# Autodesk Inventor assembly: LINEAR ACTUATOR
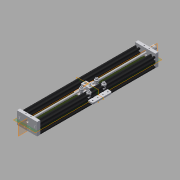
[picture p0: Inventor's stored thumbnail of the model, 180x180]
Saved by Autodesk Inventor 2016 (Build 200138000, 138)
## iProperties
Created: 2023-12-03
Part Number: LINEAR ACTUATOR
Document SubType Name: Assembly
Designer: Riskinova Oktavia
Author: Riskinova Oktavia
## Documents named in this file (33)
- D:\PROJECT NOVA 2021-2022\PBLMK-041\NEW KONSEP\LINEAR ACTUATOR.iam
- D:\PROJECT NOVA 2021-2022\PBLMK-041\PBLMK-041\Solid33.ipt
- D:\PROJECT NOVA 2021-2022\PBLMK-041\PBLMK-041\Solid45.ipt
- D:\PROJECT NOVA 2021-2022\PBLMK-041\PBLMK-041\Solid39.ipt
- D:\PROJECT NOVA 2021-2022\PBLMK-041\PBLMK-041\Solid41.ipt
- D:\PROJECT NOVA 2021-2022\PBLMK-041\PBLMK-041\Solid43.ipt
- D:\PROJECT NOVA 2021-2022\PBLMK-041\PBLMK-041\Solid44.ipt
- D:\PROJECT NOVA 2021-2022\PBLMK-041\PBLMK-041\Solid57.ipt
- D:\PROJECT NOVA 2021-2022\PBLMK-041\PBLMK-041\Solid58.ipt
- D:\PROJECT NOVA 2021-2022\PBLMK-041\PBLMK-041\Solid31.ipt
- D:\PROJECT NOVA 2021-2022\PBLMK-041\PBLMK-041\Solid32.ipt
- D:\PROJECT NOVA 2021-2022\PBLMK-041\PBLMK-041\Solid1.ipt
- D:\PROJECT NOVA 2021-2022\PBLMK-041\PBLMK-041\Solid53.ipt
- D:\PROJECT NOVA 2021-2022\PBLMK-041\PBLMK-041\Solid54.ipt
- D:\PROJECT NOVA 2021-2022\PBLMK-041\PBLMK-041\Solid55.ipt
- D:\PROJECT NOVA 2021-2022\PBLMK-041\PBLMK-041\Solid56.ipt
- D:\PROJECT NOVA 2021-2022\PBLMK-041\PBLMK-041\Solid49.ipt
- D:\PROJECT NOVA 2021-2022\PBLMK-041\PBLMK-041\Solid16.ipt
- D:\PROJECT NOVA 2021-2022\PBLMK-041\PBLMK-041\Solid15.ipt
- D:\PROJECT NOVA 2021-2022\PBLMK-041\PBLMK-041\Solid14.ipt
- D:\PROJECT NOVA 2021-2022\PBLMK-041\PBLMK-041\Solid13.ipt
- D:\PROJECT NOVA 2021-2022\PBLMK-041\PBLMK-041\Solid12.ipt
- D:\PROJECT NOVA 2021-2022\PBLMK-041\PBLMK-041\Solid11.ipt
- D:\PROJECT NOVA 2021-2022\PBLMK-041\PBLMK-041\Solid10.ipt
- D:\PROJECT NOVA 2021-2022\PBLMK-041\PBLMK-041\Solid64.ipt
- D:\PROJECT NOVA 2021-2022\PBLMK-041\PBLMK-041\Solid63.ipt
- D:\PROJECT NOVA 2021-2022\PBLMK-041\PBLMK-041\Solid62.ipt
- D:\PROJECT NOVA 2021-2022\PBLMK-041\PBLMK-041\Solid61.ipt
- D:\PROJECT NOVA 2021-2022\PBLMK-041\PBLMK-041\Solid46.ipt
- D:\PROJECT NOVA 2021-2022\PBLMK-041\PBLMK-041\Solid42.ipt
- D:\PROJECT NOVA 2021-2022\PBLMK-041\PBLMK-041\Solid40.ipt
- D:\PROJECT NOVA 2021-2022\PBLMK-041\PBLMK-041\Solid38.ipt
- D:\PROJECT NOVA 2021-2022\PBLMK-041\PBLMK-041\Solid34.ipt
## Components (59 placed, 32 different names)
1. Solid33:1
2. Solid45:1 — Flush:5
3. Solid39:1
4. Solid41:1
5. Solid43:1
6. Solid44:1 — Mate:94, Mate:95, Mate:96, Mate:97
7. Solid57:1
8. Solid58:1
9. Solid31:1
10. Solid32:1 — Flush:5
11. Solid1:1
12. Solid53:1
13. Solid54:1
14. Solid55:1
15. Solid56:1
16. Solid49:1
17. Solid16:1
18. Solid15:1
19. Solid14:1
20. Solid13:1
21. Solid12:1
22. Solid11:1
23. Solid10:1
24. Solid64:1
25. Solid63:1
26. Solid62:1
27. Solid61:1
28. Solid46:1
29. Solid42:1
30. Solid40:1
31. Solid38:1
32. Solid34:1
33. Solid49:2
34. Solid16:2
35. Solid15:2
36. Solid14:2
37. Solid13:2
38. Solid12:2
39. Solid11:2
40. Solid10:2
41. Solid49:3
42. Solid16:3
43. Solid15:3
44. Solid14:3
45. Solid13:3
46. Solid12:3
47. Solid11:3
48. Solid10:3
49. Solid49:4
50. Solid16:4
51. Solid15:4
52. Solid14:4
53. Solid13:4
54. Solid12:4
55. Solid11:4
56. Solid10:4
57. Solid1:2
58. Solid58:2 — Mate:94, Mate:96
59. Solid58:3 — Mate:95, Mate:97
## Relationships (111: Mate 91, RevoluteJoint 16, Flush 4)
- [Mate]: Solid33:1 ↔ Solid31:1
- [Mate]: Solid45:1 ↔ Solid31:1
- [Mate]: Solid31:1 ↔ Solid54:1
- [Mate]: Solid31:1 ↔ Solid53:1
- [Mate]: Solid54:1 ↔ Solid55:1
- [Mate]: Solid53:1 ↔ Solid56:1
- [Mate]: Solid31:1 ↔ Solid56:1
- [Mate]: Solid31:1 ↔ Solid55:1
- [Mate]: Solid32:1 ↔ Solid53:1
- [Mate]: Solid32:1 ↔ Solid54:1
- [RevoluteJoint]: Solid16:1 ↔ Solid14:1
- [Mate]: Solid14:1 ↔ Solid12:1
- [Mate]: Solid14:1 ↔ Solid13:1
- [Mate]: Solid16:1 ↔ Solid11:1
- [RevoluteJoint]: Solid14:1 ↔ Solid13:1
- [Mate]: Solid15:1 ↔ Solid13:1
- [RevoluteJoint]: Solid15:1 ↔ Solid13:1
- [RevoluteJoint]: Solid15:1 ↔ Solid12:1
- [Mate]: Solid12:1 ↔ Solid10:1
- [Mate]: Solid49:1 ↔ Solid15:1
- [Mate]: Solid16:1 ↔ Solid11:1
- [Mate] (2 mm): Solid49:1 ↔ Solid10:1
- [Mate]: Solid12:1 ↔ Solid10:1
- [RevoluteJoint]: Solid16:2 ↔ Solid14:2
- [Mate]: Solid14:2 ↔ Solid12:2
- [Mate]: Solid14:2 ↔ Solid13:2
- [Mate]: Solid16:2 ↔ Solid11:2
- [RevoluteJoint]: Solid14:2 ↔ Solid13:2
- [Mate]: Solid15:2 ↔ Solid13:2
- [RevoluteJoint]: Solid15:2 ↔ Solid13:2
- [RevoluteJoint]: Solid15:2 ↔ Solid12:2
- [Mate]: Solid12:2 ↔ Solid10:2
- [Mate]: Solid49:2 ↔ Solid15:2
- [Mate]: Solid16:2 ↔ Solid11:2
- [Mate] (2 mm): Solid49:2 ↔ Solid10:2
- [Mate]: Solid12:2 ↔ Solid10:2
- [RevoluteJoint]: Solid16:3 ↔ Solid14:3
- [Mate]: Solid14:3 ↔ Solid12:3
- [Mate]: Solid14:3 ↔ Solid13:3
- [Mate]: Solid16:3 ↔ Solid11:3
- [RevoluteJoint]: Solid14:3 ↔ Solid13:3
- [Mate]: Solid15:3 ↔ Solid13:3
- [RevoluteJoint]: Solid15:3 ↔ Solid13:3
- [RevoluteJoint]: Solid15:3 ↔ Solid12:3
- [Mate]: Solid12:3 ↔ Solid10:3
- [Mate]: Solid49:3 ↔ Solid15:3
- [Mate]: Solid16:3 ↔ Solid11:3
- [Mate] (2 mm): Solid49:3 ↔ Solid10:3
- [Mate]: Solid12:3 ↔ Solid10:3
- [RevoluteJoint]: Solid16:4 ↔ Solid14:4
- [Mate]: Solid14:4 ↔ Solid12:4
- [Mate]: Solid14:4 ↔ Solid13:4
- [Mate]: Solid16:4 ↔ Solid11:4
- [RevoluteJoint]: Solid14:4 ↔ Solid13:4
- [Mate]: Solid15:4 ↔ Solid13:4
- [RevoluteJoint]: Solid15:4 ↔ Solid13:4
- [RevoluteJoint]: Solid15:4 ↔ Solid12:4
- [Mate]: Solid12:4 ↔ Solid10:4
- [Mate]: Solid49:4 ↔ Solid15:4
- [Mate]: Solid16:4 ↔ Solid11:4
- [Mate] (2 mm): Solid49:4 ↔ Solid10:4
- [Mate]: Solid12:4 ↔ Solid10:4
- [Mate]: Solid32:1 ↔ Solid10:1
- [Mate]: Solid32:1 ↔ Solid49:1
- [Mate]: Solid32:1 ↔ Solid49:2
- [Mate]: Solid32:1 ↔ Solid49:2
- [Mate]: Solid32:1 ↔ Solid49:3
- [Mate]: Solid32:1 ↔ Solid49:4
- [Mate]: Solid32:1 ↔ Solid49:3
- [Mate]: Solid32:1 ↔ Solid49:4
- [Mate]: Solid54:1 ↔ Solid1:2
- [Mate]: Solid1:1 ↔ Solid53:1
- [Mate]: Solid32:1 ↔ Solid1:1
- [Mate]: Solid32:1 ↔ Solid1:2
- [Mate]: Solid31:1 ↔ Solid1:1
- [Mate]: Solid33:1 ↔ Solid46:1
- [Mate]: Solid33:1 ↔ Solid34:1
- [Mate]: Solid46:1 ↔ Solid34:1
- [Flush]: Solid33:1 ↔ Solid34:1
- [Mate]: Solid46:1 ↔ Solid42:1
- [Mate]: Solid33:1 ↔ Solid40:1
- [Mate]: Solid42:1 ↔ Solid40:1
- [Mate]: Solid33:1 ↔ Solid38:1
- [Mate]: Solid40:1 ↔ Solid38:1
- [Mate]: Solid45:1 ↔ Solid46:1
- [Flush]: Solid45:1 ↔ Solid46:1
- [Mate]: Solid33:1 ↔ Solid39:1
- [Mate]: Solid33:1 ↔ Solid43:1
- [Mate]: Solid33:1 ↔ Solid41:1
- [Mate]: Solid39:1 ↔ Solid41:1
- [Mate]: Solid41:1 ↔ Solid43:1
- [Mate]: Solid45:1 ↔ Solid44:1
- [Flush]: Solid45:1 ↔ Solid44:1
- [Mate]: Solid43:1 ↔ Solid44:1
- [Mate]: Solid44:1 ↔ Solid57:1
- [Mate]: Solid44:1 ↔ Solid58:1
- [Mate]: Solid44:1 ↔ Solid57:1
- [Mate]: Solid44:1 ↔ Solid58:1
- [Mate]: Solid61:1 ↔ Solid46:1
- [Mate]: Solid62:1 ↔ Solid46:1
- [Mate]: Solid63:1 ↔ Solid46:1
- [Mate]: Solid64:1 ↔ Solid46:1
- [Mate]: Solid61:1 ↔ Solid46:1
- [Mate]: Solid63:1 ↔ Solid46:1
- [Mate]: Solid64:1 ↔ Solid46:1
- [Mate]: Solid62:1 ↔ Solid46:1
- Flush:5: Solid45:1 ↔ Solid32:1
- Mate:94: Solid44:1 ↔ Solid58:2
- Mate:95: Solid44:1 ↔ Solid58:3
- Mate:96: Solid44:1 ↔ Solid58:2
- Mate:97: Solid44:1 ↔ Solid58:3
## Named parameters: d59_d24 = -74.535325 deg, d60_d25 = 0 mm, d61_d26 = 0 mm, d62_d27 = 0 mm, d63_d28 = 2 mm, d64_d29 = 0 mm, d65_d13 = 0 mm, d66_d14 = 22.114192 deg, d67_d15 = 0 mm, d68_d16 = 0 mm, d69_d17 = 0 mm, d70_d18 = 0 mm, d71_d19 = -0.146419 deg, d72_d20 = 0 mm, d73_d21 = 0 mm, d74_d22 = 33.946951 deg, d75_d23 = 0 mm, d76_d24 = 108.349826 deg, d77_d25 = 0 mm, d78_d26 = 0 mm, d79_d27 = 0 mm, d80_d28 = 2 mm, d231_d28 = 2 mm, d243_d1 = 0 mm, d244_d2 = 0 mm, d246_d4 = 0 mm, d247_d5 = 0 mm, d115_d114 = 0 mm, d53_d115 = 0 mm, d54_d116 = 0 mm, d57_d119 = 0 mm, d58_d120 = 0 mm, d61_d123 = 0 mm, d62_d124 = 0 mm, d63_d125 = 0 mm, d64_d126 = 0 mm, d65_d127 = 0 mm, d66_d128 = 0 mm, d67_d103 = 0 mm, d68_d104 = 0 mm, d132_d105 = 0 mm, d133_d106 = 0 mm, d134_d107 = 0 mm, d135_d108 = 0 mm, d73_d109 = 0 mm, d75_d112 = 0 mm, d76_d113 = 0 mm, d77_d91 = 0 mm, d141_d92 = 0 mm, d142_d93 = 0 mm, d143_d94 = 0 mm, d144_d95 = 0 mm, d82_d96 = 0 mm, d83_d97 = 0 mm, d84_d98 = 0 mm, d85_d99 = 0 mm, d149_d100 = 0 mm, d87_d101 = 0 mm, d151_d102 = 0 mm, d152_d81 = 0 mm, d153_d82 = 0 mm, d154_d83 = 0 mm, d155_d84 = 0 mm, d156_d85 = 0 mm, d162_d29 = 0 mm, d30_d29 = 0 mm, d31_d13 = 0 mm, d32_d14 = -2.890225 deg, d33_d15 = 0 mm, d34_d16 = 0 mm, d35_d17 = 0 mm, d36_d18 = 0 mm, d37_d19 = 0.171516 deg, d38_d20 = 0 mm, d39_d21 = 0 mm, d40_d22 = -178.30437 deg, d41_d23 = 0 mm, d42_d24 = -108.403435 deg, d43_d25 = 0 mm, d44_d26 = 0 mm, d45_d27 = 0 mm, d46_d28 = 2 mm, d47_d29 = 0 mm, d48_d13 = 0 mm, d49_d14 = -9.812675 deg, d50_d15 = 0 mm, d51_d16 = 0 mm, d52_d17 = 0 mm, d53_d18 = 0 mm, d54_d19 = 0.100861 deg, d55_d20 = 0 mm, d56_d21 = 0 mm, d57_d22 = 172.102217 deg, d58_d23 = 0 mm
